# Autodesk Inventor assembly: Assembly1
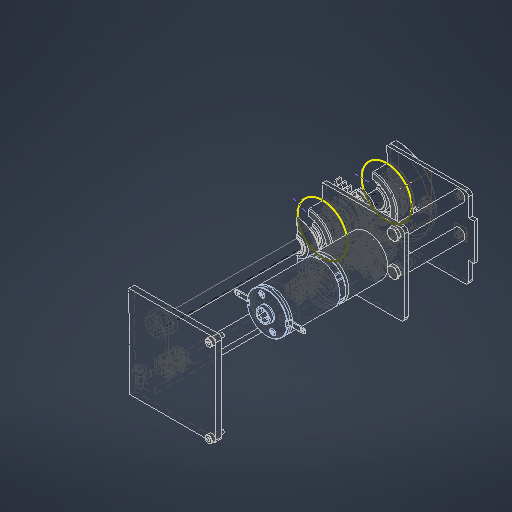
[picture p0: Inventor's stored thumbnail of the model, 512x512]
Saved by Autodesk Inventor 2026.1 (Build 301233020, 233B)
## iProperties
Created: 2026-02-25
Part Number: Assembly1
Document SubType Name: Assembly
Designer: Jan
Author: Jan
## Documents named in this file (39)
- C:\Users\Jan\OneDrive\Pulpit\Ainventor-ZNL\Assembly1.iam
- C:\Users\Jan\OneDrive\Pulpit\Ainventor-ZNL\czesci\motor-and-drive\motor-and-drive\motor-and-drive.iam
- C:\Users\Jan\OneDrive\Pulpit\Ainventor-ZNL\czesci\płyta silnika.ipt
- C:\Users\Jan\OneDrive\Pulpit\Ainventor-ZNL\czesci\Spur Gears1.iam
- C:\Users\Jan\OneDrive\Pulpit\Ainventor-ZNL\czesci\619_9.iam
- C:\Users\Jan\OneDrive\Pulpit\Ainventor-ZNL\czesci\tuleja łożyska.ipt
- C:\Users\Jan\OneDrive\Pulpit\Ainventor-ZNL\czesci\ściana.ipt
- C:\Users\Jan\OneDrive\Pulpit\Ainventor-ZNL\czesci\Compress Spring11.ipt
- C:\Users\Jan\OneDrive\Pulpit\Ainventor-ZNL\czesci\tarcza sprzęgła.ipt
- C:\Users\Jan\OneDrive\Pulpit\Ainventor-ZNL\czesci\popychacz.ipt
- C:\Users\Jan\OneDrive\Pulpit\Ainventor-ZNL\czesci\nakrętka.ipt
- C:\Users\Jan\OneDrive\Documents\Inventor\Content Center Files\R2026\en-US\DIN 471(1)\DIN 471 - 9x1.ipt
- C:\Users\Jan\OneDrive\Documents\Inventor\Content Center Files\R2026\en-US\DIN 472(1)\DIN 472 - 21 x 1.ipt
- C:\Users\Jan\OneDrive\Documents\Inventor\Content Center Files\R2026\en-US\D-Sub Male Crimp\D-Sub Male Crimp 15CKT.ipt
- C:\Users\Jan\OneDrive\Documents\Inventor\Content Center Files\R2026\en-US\DIN 471(1)\DIN 471 - 11x1.ipt
- C:\Users\Jan\OneDrive\Pulpit\Ainventor-ZNL\czesci\podkładka-sprężyny.ipt
- C:\Users\Jan\OneDrive\Pulpit\Ainventor-ZNL\czesci\tarcza sprzęgła 2.ipt
- C:\Users\Jan\OneDrive\Documents\Inventor\Content Center Files\R2026\en-US\DIN 913\DIN 913 - M2 x 3.ipt
- C:\Users\Jan\OneDrive\Pulpit\Ainventor-ZNL\czesci\słupek.ipt
- C:\Users\Jan\OneDrive\Documents\Inventor\Content Center Files\R2026\en-US\ISO 4762(1)\DIN EN ISO 4762 - M3 x 5.ipt
- C:\Users\Jan\OneDrive\Documents\Inventor\Content Center Files\R2026\en-US\ISO 4017(1)\ISO 4017 - M3 x 8 - ISO.ipt
- C:\Users\Jan\OneDrive\Pulpit\Ainventor-ZNL\czesci\obudowa.ipt
- C:\Users\Jan\OneDrive\Pulpit\Ainventor-ZNL\czesci\SS0750301F040P1A\SS0750301F040P1A\SS0750301F040P1A.ipt
- C:\Users\Jan\OneDrive\Documents\Inventor\Content Center Files\R2026\en-US\ISO 4762(2)\ISO 4762 - M3 x 5ISO.ipt
- C:\Users\Jan\OneDrive\Documents\Inventor\Content Center Files\R2026\en-US\DIN 912\DIN 912 - M1.6 x 0.35 x 2.5 x 1.625.ipt
- C:\Users\Jan\OneDrive\Pulpit\Ainventor-ZNL\czesci\tarcza krańcówek.ipt
- C:\Users\Jan\OneDrive\Documents\Inventor\Content Center Files\R2026\en-US\ISO 4032(2)\ISO 4032 - M6 - ISO.ipt
- C:\Users\Jan\OneDrive\Pulpit\Ainventor-ZNL\czesci\szyna.ipt
- C:\Users\Jan\OneDrive\Pulpit\Ainventor-ZNL\czesci\kołmierz.ipt
- C:\Users\Jan\OneDrive\Documents\Inventor\Content Center Files\R2026\en-US\ISO 4762(2)\ISO 4762 - M3 x 8ISO.ipt
- C:\Users\Jan\OneDrive\Pulpit\Ainventor-ZNL\czesci\płytka złącza.ipt
- C:\Users\Jan\OneDrive\Pulpit\Ainventor-ZNL\czesci\HEDS9100\HEDS9100\HEDS9100.ipt
- C:\Users\Jan\OneDrive\Pulpit\Ainventor-ZNL\czesci\Tarcza impulsowa HEDS-5140.ipt
- C:\Users\Jan\OneDrive\Documents\Inventor\Content Center Files\R2026\en-US\ISO 4762(2)\ISO 4762 - M2 x 20ISO.ipt
- C:\Users\Jan\OneDrive\Documents\Inventor\Content Center Files\R2026\en-US\ANSI B18.3(08)\ANSI B18.3 - 2-56 UNC - 0.125(24).ipt
- C:\Users\Jan\OneDrive\Pulpit\Ainventor-ZNL\czesci\ściana tylna.ipt
- C:\Users\Jan\OneDrive\Documents\Inventor\Content Center Files\R2026\en-US\ISO 4762(2)\ISO 4762 - M3 x 6ISO.ipt
- C:\Users\Jan\OneDrive\Documents\Inventor\Content Center Files\R2026\en-US\ISO 4762(2)\ISO 4762 - M2 x 6ISO.ipt
- C:\Users\Jan\OneDrive\Documents\Inventor\Content Center Files\R2026\en-US\ISO 4762(2)\ISO 4762 - M1.6 x 8ISO.ipt
## Components (64 placed, 38 different names)
1. motor-and-drive:1 [sub-assembly] — Mate:5, Mate:12, Mate:13, Mate:14, Angle:3, Angle:7, Angle:8, Angle:9
2. płyta silnika:1 — Mate:5, Mate:14, Mate:53, Mate:54, Angle:9, Mate:64, Mate:65, Mate:66, Mate:67, Mate:68, Mate:70, Mate:71, Mate:72, Mate:73, Mate:74, Mate:75, Mate:83, Mate:85, Mate:107, Mate:108, Mate:109, Mate:110, Mate:113, Mate:114, Mate:132, Mate:133, Angle:18
3. Spur Gears:1 [sub-assembly] — Mate:12, Mate:13, Angle:3, Mate:56, Mate:59, Mate:63, Angle:10
4. 619_9:1 [sub-assembly] — Flush:8, Mate:23
5. 619_9:2 [sub-assembly] — Mate:34, Mate:35, Mate:43
6. tuleja łożyska:1 — Insert:1, Insert:2, Mate:34, Flush:16, Mate:80
7. tuleja łożyska:2 — Flush:8, Mate:23, Insert:4, Mate:40, Mate:41, Mate:54, Mate:81, Mate:131
8. ściana:1 — Mate:61, Angle:8, Mate:69, Mate:86, Mate:87, Flush:17, Mate:104, Mate:105, Mate:106, Mate:111, Mate:112
9. Compress Spring:1 — Flush:11, Flush:12, Mate:46, Flush:14, Angle:11
10. tarcza sprzęgła:1 — Flush:14, Mate:51, Flush:15, Angle:5, Mate:56, Mate:57
11. popychacz:1 — Flush:16, Angle:5, Mate:53, Mate:55, Mate:58, Mate:61, Angle:10, Mate:80, Mate:81, Mate:90, Angle:12, Mate:91, Mate:92, Mate:126
12. nakrętka:1 — Mate:28, Mate:29, Insert:3, Mate:46, Mate:55, Mate:57, Mate:78, Flush:18, Flush:19
13. DIN 471 9x1:2 — Mate:28, Mate:29, Mate:43
14. DIN 472 21 x 1:1 — Insert:1, Mate:135
15. DIN 472 21 x 1:2 — Insert:2, Mate:35, Mate:135
16. D-Sub Male Crimp D-Sub Male Crimp 15CKT:1 — Angle:11, Mate:88, Mate:89, Mate:119, Mate:120, Mate:121, Mate:122
17. DIN 471 11x1:1 — Insert:3, Mate:39, Mate:76, Mate:77
18. podkładka-sprężyny:1 — Mate:39, Flush:13, Mate:76, Mate:77, Mate:78
19. DIN 472 21 x 1:3 — Insert:4
20. DIN 472 21 x 1:4 — Mate:40, Mate:41
21. DIN 912 - replaced by DIN EN ISO 4762 M1.6 x 2.5:1 — Mate:51, Flush:15, Flush:18
22. tarcza sprzęgła 2:1 — Mate:58, Mate:59
23. DIN 913 M2 x 3:1 — Mate:63, Angle:7
24. słupek:1 — Mate:66, Mate:67, Mate:68, Mate:69, Mate:82
25. słupek:2 — Mate:64, Mate:65, Mate:84
26. DIN EN ISO 4762 M3 x 5:1 — Mate:70, Mate:71
27. DIN EN ISO 4762 M3 x 5:2 — Mate:72, Mate:73
28. DIN EN ISO 4762 M3 x 5:3 — Mate:74, Mate:75
29. ISO 4017 M3 x 8:1 — Mate:82, Mate:83
30. ISO 4017 M3 x 8:2 — Mate:84, Mate:85
31. obudowa:1 — Mate:86, Mate:87, Flush:17, Mate:88, Mate:89, Mate:98, Mate:99, Angle:15, Mate:123, Mate:124, Mate:125, Mate:136, Mate:137, Mate:138, Mate:139, Mate:141, Mate:143, Mate:145
32. SS0750301F040P1A:1 — Mate:117, Mate:118, Angle:17, Insert:10, Insert:12
33. SS0750301F040P1A:2 — Mate:115, Angle:16, Mate:116, Insert:9, Mate:147, Mate:148
34. ISO 4762 M3 x 8:1 — Mate:119, Mate:121
35. ISO 4762 M3 x 8:2 — Mate:120, Mate:122
36. tarcza krańcówek:1 — Mate:90, Angle:12, Mate:91, Mate:93
37. ISO 4032 M6:1 — Mate:92, Mate:93
38. szyna:1 — Mate:98, Mate:99, Angle:15, Mate:100, Mate:101, Mate:102, Mate:103, Mate:115, Angle:16, Mate:116, Mate:117, Mate:118, Angle:17
39. ISO 4762 M3 x 6:1 — Mate:102, Mate:103
40. ISO 4762 M3 x 6:2 — Mate:100, Mate:101
41. kołmierz:1 — Mate:104, Mate:105, Mate:106, Insert:5, Insert:6
42. ISO 4762 M3 x 5:5 — Insert:5
43. ISO 4762 M3 x 5:6 — Insert:6
44. ISO 4017 M3 x 8:3 — Mate:108, Mate:110
45. ISO 4017 M3 x 8:4 — Mate:107, Mate:109
46. słupek:3 — Mate:111, Mate:113
47. słupek:4 — Mate:112, Mate:114
48. płytka złącza:1 — Mate:123, Mate:124, Mate:125, Insert:7, Insert:8
49. HEDS9100:1 — Mate:127, Mate:128, Mate:129, Mate:130, Mate:131
50. Tarcza impulsowa HEDS-5140:1 — Mate:126, Flush:19, Angle:18, Mate:134
51. ISO 4762 M2 x 20:1 — Mate:127, Mate:129, Mate:132
52. ISO 4762 M2 x 20:2 — Mate:128, Mate:130, Mate:133
53. Hexagon Socket Set Screw - Flat Point - Inch 2-56 UNC x 0.125:1 — Mate:134
54. ściana tylna:1 — Mate:136, Mate:137, Mate:138, Mate:140, Mate:142, Mate:144, Mate:146
55. ISO 4762 M3 x 5:7 — Insert:7
56. ISO 4762 M3 x 5:8 — Insert:8
57. ISO 4762 M2 x 6:1 — Mate:139, Mate:140
58. ISO 4762 M2 x 6:2 — Mate:141, Mate:142
59. ISO 4762 M2 x 6:3 — Mate:143, Mate:144
60. ISO 4762 M2 x 6:4 — Mate:145, Mate:146
61. ISO 4762 M1.6 x 8:1 — Insert:9
62. ISO 4762 M1.6 x 8:2 — Mate:147, Mate:148
63. ISO 4762 M1.6 x 8:3 — Insert:10
64. ISO 4762 M1.6 x 8:4 — Insert:12
## Relationships (137: Mate 104, Angle 12, Insert 11, Flush 10)
- Mate:5: motor-and-drive:1 ↔ płyta silnika:1
- Mate:12 (-8.5 mm): motor-and-drive:1 ↔ Spur Gears:1
- Mate:13: motor-and-drive:1 ↔ Spur Gears:1
- Mate:14: motor-and-drive:1 ↔ płyta silnika:1
- Flush:8 (-2 mm): 619_9:1 ↔ tuleja łożyska:2
- Mate:23: 619_9:1 ↔ tuleja łożyska:2
- Mate:28: nakrętka:1 ↔ DIN 471 9x1:2
- Mate:29: nakrętka:1 ↔ DIN 471 9x1:2
- Insert:1: tuleja łożyska:1 ↔ DIN 472 21 x 1:1
- Insert:2: tuleja łożyska:1 ↔ DIN 472 21 x 1:2
- Mate:34: 619_9:2 ↔ tuleja łożyska:1
- Mate:35: 619_9:2 ↔ DIN 472 21 x 1:2
- Insert:3: nakrętka:1 ↔ DIN 471 11x1:1
- Mate:39: DIN 471 11x1:1 ↔ podkładka-sprężyny:1
- Angle:3 (0 deg): motor-and-drive:1 ↔ Spur Gears:1
- Insert:4: tuleja łożyska:2 ↔ DIN 472 21 x 1:3
- Mate:40: tuleja łożyska:2 ↔ DIN 472 21 x 1:4
- Mate:41: tuleja łożyska:2 ↔ DIN 472 21 x 1:4
- Mate:43: 619_9:2 ↔ DIN 471 9x1:2
- Flush:11 (-4 mm): Compress Spring:1
- Flush:12 (4 mm): Compress Spring:1
- Flush:13: podkładka-sprężyny:1
- Mate:46: Compress Spring:1 ↔ nakrętka:1
- Flush:14: Compress Spring:1 ↔ tarcza sprzęgła:1
- Mate:51: tarcza sprzęgła:1 ↔ DIN 912 - replaced by DIN EN ISO 4762 M1.6 x 2.5:1
- Flush:15 (0.4 mm): tarcza sprzęgła:1 ↔ DIN 912 - replaced by DIN EN ISO 4762 M1.6 x 2.5:1
- Flush:16: tuleja łożyska:1 ↔ popychacz:1
- Angle:5 (0 deg): tarcza sprzęgła:1 ↔ popychacz:1
- Mate:53: płyta silnika:1 ↔ popychacz:1
- Mate:54: płyta silnika:1 ↔ tuleja łożyska:2
- Mate:55: popychacz:1 ↔ nakrętka:1
- Mate:56: Spur Gears:1 ↔ tarcza sprzęgła:1
- Mate:57: tarcza sprzęgła:1 ↔ nakrętka:1
- Mate:58: popychacz:1 ↔ tarcza sprzęgła 2:1
- Mate:59: Spur Gears:1 ↔ tarcza sprzęgła 2:1
- Mate:61: ściana:1 ↔ popychacz:1
- Mate:63: Spur Gears:1 ↔ DIN 913 M2 x 3:1
- Angle:7 (0 deg): motor-and-drive:1 ↔ DIN 913 M2 x 3:1
- Angle:8 (0 deg): motor-and-drive:1 ↔ ściana:1
- Angle:9 (0 deg): motor-and-drive:1 ↔ płyta silnika:1
- Mate:64: płyta silnika:1 ↔ słupek:2
- Mate:65: płyta silnika:1 ↔ słupek:2
- Mate:66: płyta silnika:1 ↔ słupek:1
- Mate:67: płyta silnika:1 ↔ słupek:1
- Mate:68: płyta silnika:1 ↔ słupek:1
- Angle:10 (0 deg): Spur Gears:1 ↔ popychacz:1
- Mate:69: ściana:1 ↔ słupek:1
- Mate:70: płyta silnika:1 ↔ DIN EN ISO 4762 M3 x 5:1
- Mate:71: płyta silnika:1 ↔ DIN EN ISO 4762 M3 x 5:1
- Mate:72: płyta silnika:1 ↔ DIN EN ISO 4762 M3 x 5:2
- Mate:73: płyta silnika:1 ↔ DIN EN ISO 4762 M3 x 5:2
- Mate:74: płyta silnika:1 ↔ DIN EN ISO 4762 M3 x 5:3
- Mate:75: płyta silnika:1 ↔ DIN EN ISO 4762 M3 x 5:3
- Mate:76: DIN 471 11x1:1 ↔ podkładka-sprężyny:1
- Mate:77: DIN 471 11x1:1 ↔ podkładka-sprężyny:1
- Mate:78: nakrętka:1 ↔ podkładka-sprężyny:1
- Mate:80: tuleja łożyska:1 ↔ popychacz:1
- Mate:81: tuleja łożyska:2 ↔ popychacz:1
- Mate:82: słupek:1 ↔ ISO 4017 M3 x 8:1
- Mate:83 (-0.4 mm): płyta silnika:1 ↔ ISO 4017 M3 x 8:1
- Mate:84: słupek:2 ↔ ISO 4017 M3 x 8:2
- Mate:85 (-0.4 mm): płyta silnika:1 ↔ ISO 4017 M3 x 8:2
- Mate:86: ściana:1 ↔ obudowa:1
- Mate:87: ściana:1 ↔ obudowa:1
- Flush:17: ściana:1 ↔ obudowa:1
- Angle:11 (90 deg): Compress Spring:1 ↔ D-Sub Male Crimp D-Sub Male Crimp 15CKT:1
- Mate:88: D-Sub Male Crimp D-Sub Male Crimp 15CKT:1 ↔ obudowa:1
- Mate:89: D-Sub Male Crimp D-Sub Male Crimp 15CKT:1 ↔ obudowa:1
- Flush:18: nakrętka:1 ↔ DIN 912 - replaced by DIN EN ISO 4762 M1.6 x 2.5:1
- Mate:90: popychacz:1 ↔ tarcza krańcówek:1
- Angle:12 (180 deg): popychacz:1 ↔ tarcza krańcówek:1
- Mate:91: popychacz:1 ↔ tarcza krańcówek:1
- Mate:92: popychacz:1 ↔ ISO 4032 M6:1
- Mate:93: tarcza krańcówek:1 ↔ ISO 4032 M6:1
- Mate:98: obudowa:1 ↔ szyna:1
- Mate:99: obudowa:1 ↔ szyna:1
- Angle:15 (0 deg): obudowa:1 ↔ szyna:1
- Mate:100: szyna:1 ↔ ISO 4762 M3 x 6:2
- Mate:101: szyna:1 ↔ ISO 4762 M3 x 6:2
- Mate:102: szyna:1 ↔ ISO 4762 M3 x 6:1
- Mate:103: szyna:1 ↔ ISO 4762 M3 x 6:1
- Mate:104: ściana:1 ↔ kołmierz:1
- Mate:105: ściana:1 ↔ kołmierz:1
- Mate:106: ściana:1 ↔ kołmierz:1
- Insert:5: kołmierz:1 ↔ ISO 4762 M3 x 5:5
- Insert:6: kołmierz:1 ↔ ISO 4762 M3 x 5:6
- Mate:107: płyta silnika:1 ↔ ISO 4017 M3 x 8:4
- Mate:108: płyta silnika:1 ↔ ISO 4017 M3 x 8:3
- Mate:109: płyta silnika:1 ↔ ISO 4017 M3 x 8:4
- Mate:110: płyta silnika:1 ↔ ISO 4017 M3 x 8:3
- Mate:111: ściana:1 ↔ słupek:3
- Mate:112: ściana:1 ↔ słupek:4
- Mate:113: płyta silnika:1 ↔ słupek:3
- Mate:114 (-1 mm): płyta silnika:1 ↔ słupek:4
- Mate:115: SS0750301F040P1A:2 ↔ szyna:1
- Angle:16 (0 deg): SS0750301F040P1A:2 ↔ szyna:1
- Mate:116: SS0750301F040P1A:2 ↔ szyna:1
- Mate:117: SS0750301F040P1A:1 ↔ szyna:1
- Mate:118: SS0750301F040P1A:1 ↔ szyna:1
- Angle:17 (0 deg): SS0750301F040P1A:1 ↔ szyna:1
- Mate:119: D-Sub Male Crimp D-Sub Male Crimp 15CKT:1 ↔ ISO 4762 M3 x 8:1
- Mate:120: D-Sub Male Crimp D-Sub Male Crimp 15CKT:1 ↔ ISO 4762 M3 x 8:2
- Mate:121: D-Sub Male Crimp D-Sub Male Crimp 15CKT:1 ↔ ISO 4762 M3 x 8:1
- Mate:122: D-Sub Male Crimp D-Sub Male Crimp 15CKT:1 ↔ ISO 4762 M3 x 8:2
- Mate:123: obudowa:1 ↔ płytka złącza:1
- Mate:124: obudowa:1 ↔ płytka złącza:1
- Mate:125: obudowa:1 ↔ płytka złącza:1
- Mate:126: popychacz:1 ↔ Tarcza impulsowa HEDS-5140:1
- Mate:127: HEDS9100:1 ↔ ISO 4762 M2 x 20:1
- Mate:128: HEDS9100:1 ↔ ISO 4762 M2 x 20:2
- Mate:129: HEDS9100:1 ↔ ISO 4762 M2 x 20:1
- Mate:130: HEDS9100:1 ↔ ISO 4762 M2 x 20:2
- Mate:131: tuleja łożyska:2 ↔ HEDS9100:1
- Flush:19: nakrętka:1 ↔ Tarcza impulsowa HEDS-5140:1
- Mate:132: płyta silnika:1 ↔ ISO 4762 M2 x 20:1
- Mate:133: płyta silnika:1 ↔ ISO 4762 M2 x 20:2
- Angle:18 (180 deg): płyta silnika:1 ↔ Tarcza impulsowa HEDS-5140:1
- Mate:134: Tarcza impulsowa HEDS-5140:1 ↔ Hexagon Socket Set Screw - Flat Point - Inch 2-56 UNC x 0.125:1
- Mate:135: DIN 472 21 x 1:1 ↔ DIN 472 21 x 1:2
- Mate:136: obudowa:1 ↔ ściana tylna:1
- Mate:137: obudowa:1 ↔ ściana tylna:1
- Mate:138: obudowa:1 ↔ ściana tylna:1
- Insert:7: płytka złącza:1 ↔ ISO 4762 M3 x 5:7
- Insert:8: płytka złącza:1 ↔ ISO 4762 M3 x 5:8
- Mate:139: obudowa:1 ↔ ISO 4762 M2 x 6:1
- Mate:140: ściana tylna:1 ↔ ISO 4762 M2 x 6:1
- Mate:141: obudowa:1 ↔ ISO 4762 M2 x 6:2
- Mate:142: ściana tylna:1 ↔ ISO 4762 M2 x 6:2
- Mate:143: obudowa:1 ↔ ISO 4762 M2 x 6:3
- Mate:144: ściana tylna:1 ↔ ISO 4762 M2 x 6:3
- Mate:145: obudowa:1 ↔ ISO 4762 M2 x 6:4
- Mate:146: ściana tylna:1 ↔ ISO 4762 M2 x 6:4
- Insert:9: SS0750301F040P1A:2 ↔ ISO 4762 M1.6 x 8:1
- Mate:147: SS0750301F040P1A:2 ↔ ISO 4762 M1.6 x 8:2
- Mate:148: SS0750301F040P1A:2 ↔ ISO 4762 M1.6 x 8:2
- Insert:10: SS0750301F040P1A:1 ↔ ISO 4762 M1.6 x 8:3
- Insert:12: SS0750301F040P1A:1 ↔ ISO 4762 M1.6 x 8:4
